# Autodesk Inventor assembly: Drivebase AM14U4 Square 28inx28in
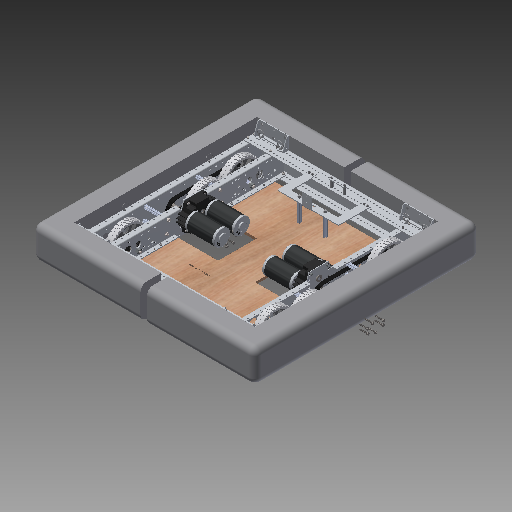
[picture p0: Inventor's stored thumbnail of the model, 512x512]
Saved by Autodesk Inventor 2018 (Build 220112000, 112)
## iProperties
Created: 2018-10-11
Part Number: Drivebase AM14U4 Square 28inx28in
Description: STEP AP214
Document SubType Name: Assembly
Designer: maste
Sending System: SolidWorks 2018
Preprocessor: SwSTEP 2.0
Title: AM14U4 Square.STEP
Revision Number: ANY
## Documents named in this file (10)
- \\studenthome\students\S-2513225\GitHub\2020CAD\Drivebase AM14U1\Main Assembly File\Drivebase AM14U4 Square 28inx28in.iam
- \\studenthome\students\S-2513225\GitHub\2020CAD\Drivebase AM14U1\Part Files\AM14U4 Square Half.iam
- \\studenthome\students\S-2513225\GitHub\2020CAD\Drivebase AM14U1\Part Files\Placeholder Belly Pan.ipt
- \\studenthome\students\S-2513225\GitHub\2020CAD\Drivebase AM14U1\Part Files\Bolts\92196A247_18-8 STAINLESS STEEL SOCKET HEAD CAP SCREW.ipt
- \\studenthome\students\S-2513225\GitHub\2020CAD\Drivebase AM14U1\Part Files\Locknuts\91831A011_TYPE 18-8 STAINLESS STL NYLON-INSERT LOCKNUT.ipt
- \\studenthome\students\S-2513225\GitHub\2020CAD\Drivebase AM14U1\Part Files\10-24 Washer.ipt
- \\studenthome\students\S-2513225\GitHub\2020CAD\Bumpers\Main Assembly File\Bumper Assembly.iam
- \\studenthome\students\S-2513225\GitHub\2020CAD\Bumpers\Part Files\95335A503_METRIC QUICK-RELEASE PIN.ipt
- \\studenthome\students\S-2513225\GitHub\2020CAD\Drivebase AM14U1\Part Files\Battery holder assembly.iam
- \\studenthome\students\S-2513225\GitHub\2020CAD\Drivebase AM14U1\Part Files\Strap mount.iam
## Components (43 placed, 10 different names)
1. AM14U4 Square Half_1 [sub-assembly] — Mate:1, Mate:2, Flush:1, Mate:3, Mate:4, Mate:5, Mate:8, Mate:9, Mate:12, Mate:13, Mate:14, Mate:15, Mate:20, Mate:21, Mate:54, Mate:55, Mate:56, Mate:57, Mate:58, Mate:66, Mate:67, Tangent:7, Tangent:8, Rotation:31, Rotation:32, Mate:72, Mate:73, Mate:74, Mate:75, Mate:76, Mate:77
2. AM14U4 Square Half_2 [sub-assembly] — Mate:1, Mate:2, Flush:1, Mate:6, Mate:7, Mate:10, Mate:11, Mate:16, Mate:17, Mate:18, Mate:19, Mate:59, Mate:60, Tangent:1, Mate:61, Tangent:2, Rotation:25, Rotation:26
3. Placeholder Belly Pan:1 — Mate:3, Mate:4, Mate:5, Mate:22, Mate:23, Mate:24, Mate:25, Mate:26, Mate:27, Mate:28, Mate:29, Rotation:1, Rotation:2, Rotation:3, Rotation:4, Rotation:5, Rotation:6, Rotation:7, Rotation:8, Rotation:9, Rotation:10, Rotation:11, Rotation:12, Rotation:13, Rotation:14, Rotation:15, Rotation:16, Mate:38, Mate:39, Mate:40, Mate:41, Mate:42, Mate:43, Mate:44, Mate:45
4. 92196A247_18-8 STAINLESS STEEL SOCKET HEAD CAP SCREW:1 — Mate:7, Mate:19, Mate:35, Rotation:5, Mate:50, Rotation:17
5. 92196A247_18-8 STAINLESS STEEL SOCKET HEAD CAP SCREW:2 — Mate:6, Mate:18, Mate:34, Rotation:7, Mate:51, Rotation:18
6. 92196A247_18-8 STAINLESS STEEL SOCKET HEAD CAP SCREW:3 — Mate:10, Mate:17, Mate:33, Rotation:9, Mate:52, Rotation:24
7. 92196A247_18-8 STAINLESS STEEL SOCKET HEAD CAP SCREW:4 — Mate:11, Mate:16, Mate:32, Rotation:11, Mate:53, Rotation:23
8. 92196A247_18-8 STAINLESS STEEL SOCKET HEAD CAP SCREW:5 — Mate:12, Mate:14, Mate:31, Rotation:13, Mate:46, Rotation:22
9. 92196A247_18-8 STAINLESS STEEL SOCKET HEAD CAP SCREW:6 — Mate:13, Mate:15, Mate:30, Rotation:15, Mate:47, Rotation:21
10. 92196A247_18-8 STAINLESS STEEL SOCKET HEAD CAP SCREW:7 — Mate:8, Mate:20, Mate:37, Rotation:1, Mate:48, Rotation:19
11. 92196A247_18-8 STAINLESS STEEL SOCKET HEAD CAP SCREW:8 — Mate:9, Mate:21, Mate:36, Rotation:3, Mate:49, Rotation:20
12. 91831A011_TYPE 18-8 STAINLESS STL NYLON-INSERT LOCKNUT:1 — Mate:42, Mate:49, Rotation:20
13. 91831A011_TYPE 18-8 STAINLESS STL NYLON-INSERT LOCKNUT:2 — Mate:43, Mate:48, Rotation:19
14. 91831A011_TYPE 18-8 STAINLESS STL NYLON-INSERT LOCKNUT:3 — Mate:44, Mate:47, Rotation:21
15. 91831A011_TYPE 18-8 STAINLESS STL NYLON-INSERT LOCKNUT:4 — Mate:45, Mate:46, Rotation:22
16. 91831A011_TYPE 18-8 STAINLESS STL NYLON-INSERT LOCKNUT:5 — Mate:41, Mate:53, Rotation:23
17. 91831A011_TYPE 18-8 STAINLESS STL NYLON-INSERT LOCKNUT:6 — Mate:40, Mate:52, Rotation:24
18. 91831A011_TYPE 18-8 STAINLESS STL NYLON-INSERT LOCKNUT:7 — Mate:39, Mate:51, Rotation:18
19. 91831A011_TYPE 18-8 STAINLESS STL NYLON-INSERT LOCKNUT:8 — Mate:38, Mate:50, Rotation:17
20. 10-24 Washer:1 — Mate:24, Mate:35, Rotation:6
21. 10-24 Washer:2 — Mate:25, Mate:34, Rotation:8
22. 10-24 Washer:3 — Mate:26, Mate:33, Rotation:10
23. 10-24 Washer:4 — Mate:27, Mate:32, Rotation:12
24. 10-24 Washer:5 — Mate:28, Mate:31, Rotation:14
25. 10-24 Washer:6 — Mate:29, Mate:30, Rotation:16
26. 10-24 Washer:7 — Mate:23, Mate:37, Rotation:2
27. 10-24 Washer:8 — Mate:22, Mate:36, Rotation:4
28. Bumper Assembly:1 [sub-assembly] — Mate:54, Mate:55, Mate:56, Mate:64, Mate:65, Mate:70, Mate:71, Tangent:5, Tangent:6, Tangent:9, Tangent:10, Rotation:29, Rotation:30, Rotation:33, Rotation:34
29. Bumper Assembly:2 [sub-assembly] — Mate:57, Mate:58, Mate:59, Mate:62, Mate:63, Mate:68, Mate:69, Tangent:3, Tangent:4, Tangent:11, Tangent:12, Rotation:27, Rotation:28, Rotation:35, Rotation:36
30. 95335A503_METRIC QUICK-RELEASE PIN:1 — Mate:62, Tangent:3, Rotation:27
31. 95335A503_METRIC QUICK-RELEASE PIN:2 — Mate:63, Tangent:4, Rotation:28
32. 95335A503_METRIC QUICK-RELEASE PIN:3 — Mate:65, Tangent:6, Rotation:30
33. 95335A503_METRIC QUICK-RELEASE PIN:4 — Mate:64, Tangent:5, Rotation:29
34. 95335A503_METRIC QUICK-RELEASE PIN:5 — Mate:71, Tangent:9, Rotation:33
35. 95335A503_METRIC QUICK-RELEASE PIN:6 — Mate:70, Tangent:10, Rotation:34
36. 95335A503_METRIC QUICK-RELEASE PIN:7 — Mate:69, Tangent:11, Rotation:35
37. 95335A503_METRIC QUICK-RELEASE PIN:8 — Mate:68, Tangent:12, Rotation:36
38. 95335A503_METRIC QUICK-RELEASE PIN:9 — Mate:61, Tangent:2, Rotation:26
39. 95335A503_METRIC QUICK-RELEASE PIN:10 — Mate:60, Tangent:1, Rotation:25
40. 95335A503_METRIC QUICK-RELEASE PIN:11 — Mate:66, Tangent:7, Rotation:31
41. 95335A503_METRIC QUICK-RELEASE PIN:12 — Mate:67, Tangent:8, Rotation:32
42. Battery holder assembly:1 [sub-assembly] — Mate:72, Mate:73, Mate:74
43. Strap mount:1 [sub-assembly] — Mate:75, Mate:76, Mate:77
## Relationships (126: Mate 77, RelateRotation 36, Tangent 12, Flush 1)
- Mate:1: AM14U4 Square Half_1 ↔ AM14U4 Square Half_2
- Mate:2: AM14U4 Square Half_1 ↔ AM14U4 Square Half_2
- Flush:1: AM14U4 Square Half_1 ↔ AM14U4 Square Half_2
- Mate:3: AM14U4 Square Half_1 ↔ Placeholder Belly Pan:1
- Mate:4: AM14U4 Square Half_1 ↔ Placeholder Belly Pan:1
- Mate:5: AM14U4 Square Half_1 ↔ Placeholder Belly Pan:1
- Mate:6: AM14U4 Square Half_2 ↔ 92196A247_18-8 STAINLESS STEEL SOCKET HEAD CAP SCREW:2
- Mate:7: AM14U4 Square Half_2 ↔ 92196A247_18-8 STAINLESS STEEL SOCKET HEAD CAP SCREW:1
- Mate:8: AM14U4 Square Half_1 ↔ 92196A247_18-8 STAINLESS STEEL SOCKET HEAD CAP SCREW:7
- Mate:9: AM14U4 Square Half_1 ↔ 92196A247_18-8 STAINLESS STEEL SOCKET HEAD CAP SCREW:8
- Mate:10: AM14U4 Square Half_2 ↔ 92196A247_18-8 STAINLESS STEEL SOCKET HEAD CAP SCREW:3
- Mate:11: AM14U4 Square Half_2 ↔ 92196A247_18-8 STAINLESS STEEL SOCKET HEAD CAP SCREW:4
- Mate:12: AM14U4 Square Half_1 ↔ 92196A247_18-8 STAINLESS STEEL SOCKET HEAD CAP SCREW:5
- Mate:13: AM14U4 Square Half_1 ↔ 92196A247_18-8 STAINLESS STEEL SOCKET HEAD CAP SCREW:6
- Mate:14: AM14U4 Square Half_1 ↔ 92196A247_18-8 STAINLESS STEEL SOCKET HEAD CAP SCREW:5
- Mate:15: AM14U4 Square Half_1 ↔ 92196A247_18-8 STAINLESS STEEL SOCKET HEAD CAP SCREW:6
- Mate:16: AM14U4 Square Half_2 ↔ 92196A247_18-8 STAINLESS STEEL SOCKET HEAD CAP SCREW:4
- Mate:17: AM14U4 Square Half_2 ↔ 92196A247_18-8 STAINLESS STEEL SOCKET HEAD CAP SCREW:3
- Mate:18: AM14U4 Square Half_2 ↔ 92196A247_18-8 STAINLESS STEEL SOCKET HEAD CAP SCREW:2
- Mate:19: AM14U4 Square Half_2 ↔ 92196A247_18-8 STAINLESS STEEL SOCKET HEAD CAP SCREW:1
- Mate:20: AM14U4 Square Half_1 ↔ 92196A247_18-8 STAINLESS STEEL SOCKET HEAD CAP SCREW:7
- Mate:21: AM14U4 Square Half_1 ↔ 92196A247_18-8 STAINLESS STEEL SOCKET HEAD CAP SCREW:8
- Mate:22: Placeholder Belly Pan:1 ↔ 10-24 Washer:8
- Mate:23: Placeholder Belly Pan:1 ↔ 10-24 Washer:7
- Mate:24: Placeholder Belly Pan:1 ↔ 10-24 Washer:1
- Mate:25: Placeholder Belly Pan:1 ↔ 10-24 Washer:2
- Mate:26: Placeholder Belly Pan:1 ↔ 10-24 Washer:3
- Mate:27: Placeholder Belly Pan:1 ↔ 10-24 Washer:4
- Mate:28: Placeholder Belly Pan:1 ↔ 10-24 Washer:5
- Mate:29: Placeholder Belly Pan:1 ↔ 10-24 Washer:6
- Mate:30: 92196A247_18-8 STAINLESS STEEL SOCKET HEAD CAP SCREW:6 ↔ 10-24 Washer:6
- Mate:31: 92196A247_18-8 STAINLESS STEEL SOCKET HEAD CAP SCREW:5 ↔ 10-24 Washer:5
- Mate:32: 92196A247_18-8 STAINLESS STEEL SOCKET HEAD CAP SCREW:4 ↔ 10-24 Washer:4
- Mate:33: 92196A247_18-8 STAINLESS STEEL SOCKET HEAD CAP SCREW:3 ↔ 10-24 Washer:3
- Mate:34: 92196A247_18-8 STAINLESS STEEL SOCKET HEAD CAP SCREW:2 ↔ 10-24 Washer:2
- Mate:35: 92196A247_18-8 STAINLESS STEEL SOCKET HEAD CAP SCREW:1 ↔ 10-24 Washer:1
- Mate:36: 92196A247_18-8 STAINLESS STEEL SOCKET HEAD CAP SCREW:8 ↔ 10-24 Washer:8
- Mate:37: 92196A247_18-8 STAINLESS STEEL SOCKET HEAD CAP SCREW:7 ↔ 10-24 Washer:7
- Rotation:1 [RelateRotation] (1 ul): Placeholder Belly Pan:1 ↔ 92196A247_18-8 STAINLESS STEEL SOCKET HEAD CAP SCREW:7
- Rotation:2 [RelateRotation] (1 ul): Placeholder Belly Pan:1 ↔ 10-24 Washer:7
- Rotation:3 [RelateRotation] (1 ul): Placeholder Belly Pan:1 ↔ 92196A247_18-8 STAINLESS STEEL SOCKET HEAD CAP SCREW:8
- Rotation:4 [RelateRotation] (1 ul): Placeholder Belly Pan:1 ↔ 10-24 Washer:8
- Rotation:5 [RelateRotation] (1 ul): Placeholder Belly Pan:1 ↔ 92196A247_18-8 STAINLESS STEEL SOCKET HEAD CAP SCREW:1
- Rotation:6 [RelateRotation] (1 ul): Placeholder Belly Pan:1 ↔ 10-24 Washer:1
- Rotation:7 [RelateRotation] (1 ul): Placeholder Belly Pan:1 ↔ 92196A247_18-8 STAINLESS STEEL SOCKET HEAD CAP SCREW:2
- Rotation:8 [RelateRotation] (1 ul): Placeholder Belly Pan:1 ↔ 10-24 Washer:2
- Rotation:9 [RelateRotation] (1 ul): Placeholder Belly Pan:1 ↔ 92196A247_18-8 STAINLESS STEEL SOCKET HEAD CAP SCREW:3
- Rotation:10 [RelateRotation] (1 ul): Placeholder Belly Pan:1 ↔ 10-24 Washer:3
- Rotation:11 [RelateRotation] (1 ul): Placeholder Belly Pan:1 ↔ 92196A247_18-8 STAINLESS STEEL SOCKET HEAD CAP SCREW:4
- Rotation:12 [RelateRotation] (1 ul): Placeholder Belly Pan:1 ↔ 10-24 Washer:4
- Rotation:13 [RelateRotation] (1 ul): Placeholder Belly Pan:1 ↔ 92196A247_18-8 STAINLESS STEEL SOCKET HEAD CAP SCREW:5
- Rotation:14 [RelateRotation] (1 ul): Placeholder Belly Pan:1 ↔ 10-24 Washer:5
- Rotation:15 [RelateRotation] (1 ul): Placeholder Belly Pan:1 ↔ 92196A247_18-8 STAINLESS STEEL SOCKET HEAD CAP SCREW:6
- Rotation:16 [RelateRotation] (1 ul): Placeholder Belly Pan:1 ↔ 10-24 Washer:6
- Mate:38: Placeholder Belly Pan:1 ↔ 91831A011_TYPE 18-8 STAINLESS STL NYLON-INSERT LOCKNUT:8
- Mate:39: Placeholder Belly Pan:1 ↔ 91831A011_TYPE 18-8 STAINLESS STL NYLON-INSERT LOCKNUT:7
- Mate:40: Placeholder Belly Pan:1 ↔ 91831A011_TYPE 18-8 STAINLESS STL NYLON-INSERT LOCKNUT:6
- Mate:41: Placeholder Belly Pan:1 ↔ 91831A011_TYPE 18-8 STAINLESS STL NYLON-INSERT LOCKNUT:5
- Mate:42: Placeholder Belly Pan:1 ↔ 91831A011_TYPE 18-8 STAINLESS STL NYLON-INSERT LOCKNUT:1
- Mate:43: Placeholder Belly Pan:1 ↔ 91831A011_TYPE 18-8 STAINLESS STL NYLON-INSERT LOCKNUT:2
- Mate:44: Placeholder Belly Pan:1 ↔ 91831A011_TYPE 18-8 STAINLESS STL NYLON-INSERT LOCKNUT:3
- Mate:45: Placeholder Belly Pan:1 ↔ 91831A011_TYPE 18-8 STAINLESS STL NYLON-INSERT LOCKNUT:4
- Mate:46: 92196A247_18-8 STAINLESS STEEL SOCKET HEAD CAP SCREW:5 ↔ 91831A011_TYPE 18-8 STAINLESS STL NYLON-INSERT LOCKNUT:4
- Mate:47: 92196A247_18-8 STAINLESS STEEL SOCKET HEAD CAP SCREW:6 ↔ 91831A011_TYPE 18-8 STAINLESS STL NYLON-INSERT LOCKNUT:3
- Mate:48: 92196A247_18-8 STAINLESS STEEL SOCKET HEAD CAP SCREW:7 ↔ 91831A011_TYPE 18-8 STAINLESS STL NYLON-INSERT LOCKNUT:2
- Mate:49: 92196A247_18-8 STAINLESS STEEL SOCKET HEAD CAP SCREW:8 ↔ 91831A011_TYPE 18-8 STAINLESS STL NYLON-INSERT LOCKNUT:1
- Mate:50: 92196A247_18-8 STAINLESS STEEL SOCKET HEAD CAP SCREW:1 ↔ 91831A011_TYPE 18-8 STAINLESS STL NYLON-INSERT LOCKNUT:8
- Mate:51: 92196A247_18-8 STAINLESS STEEL SOCKET HEAD CAP SCREW:2 ↔ 91831A011_TYPE 18-8 STAINLESS STL NYLON-INSERT LOCKNUT:7
- Mate:52: 92196A247_18-8 STAINLESS STEEL SOCKET HEAD CAP SCREW:3 ↔ 91831A011_TYPE 18-8 STAINLESS STL NYLON-INSERT LOCKNUT:6
- Mate:53: 92196A247_18-8 STAINLESS STEEL SOCKET HEAD CAP SCREW:4 ↔ 91831A011_TYPE 18-8 STAINLESS STL NYLON-INSERT LOCKNUT:5
- Rotation:17 [RelateRotation] (1 ul): 92196A247_18-8 STAINLESS STEEL SOCKET HEAD CAP SCREW:1 ↔ 91831A011_TYPE 18-8 STAINLESS STL NYLON-INSERT LOCKNUT:8
- Rotation:18 [RelateRotation] (1 ul): 92196A247_18-8 STAINLESS STEEL SOCKET HEAD CAP SCREW:2 ↔ 91831A011_TYPE 18-8 STAINLESS STL NYLON-INSERT LOCKNUT:7
- Rotation:19 [RelateRotation] (1 ul): 92196A247_18-8 STAINLESS STEEL SOCKET HEAD CAP SCREW:7 ↔ 91831A011_TYPE 18-8 STAINLESS STL NYLON-INSERT LOCKNUT:2
- Rotation:20 [RelateRotation] (1 ul): 92196A247_18-8 STAINLESS STEEL SOCKET HEAD CAP SCREW:8 ↔ 91831A011_TYPE 18-8 STAINLESS STL NYLON-INSERT LOCKNUT:1
- Rotation:21 [RelateRotation] (1 ul): 92196A247_18-8 STAINLESS STEEL SOCKET HEAD CAP SCREW:6 ↔ 91831A011_TYPE 18-8 STAINLESS STL NYLON-INSERT LOCKNUT:3
- Rotation:22 [RelateRotation] (1 ul): 92196A247_18-8 STAINLESS STEEL SOCKET HEAD CAP SCREW:5 ↔ 91831A011_TYPE 18-8 STAINLESS STL NYLON-INSERT LOCKNUT:4
- Rotation:23 [RelateRotation] (1 ul): 92196A247_18-8 STAINLESS STEEL SOCKET HEAD CAP SCREW:4 ↔ 91831A011_TYPE 18-8 STAINLESS STL NYLON-INSERT LOCKNUT:5
- Rotation:24 [RelateRotation] (1 ul): 92196A247_18-8 STAINLESS STEEL SOCKET HEAD CAP SCREW:3 ↔ 91831A011_TYPE 18-8 STAINLESS STL NYLON-INSERT LOCKNUT:6
- Mate:54: AM14U4 Square Half_1 ↔ Bumper Assembly:1
- Mate:55: AM14U4 Square Half_1 ↔ Bumper Assembly:1
- Mate:56: AM14U4 Square Half_1 ↔ Bumper Assembly:1
- Mate:57: AM14U4 Square Half_1 ↔ Bumper Assembly:2
- Mate:58: AM14U4 Square Half_1 ↔ Bumper Assembly:2
- Mate:59: AM14U4 Square Half_2 ↔ Bumper Assembly:2
- Mate:60: AM14U4 Square Half_2 ↔ 95335A503_METRIC QUICK-RELEASE PIN:10
- Tangent:1: AM14U4 Square Half_2 ↔ 95335A503_METRIC QUICK-RELEASE PIN:10
- Mate:61: AM14U4 Square Half_2 ↔ 95335A503_METRIC QUICK-RELEASE PIN:9
- Mate:62: Bumper Assembly:2 ↔ 95335A503_METRIC QUICK-RELEASE PIN:1
- Mate:63: Bumper Assembly:2 ↔ 95335A503_METRIC QUICK-RELEASE PIN:2
- Mate:64: Bumper Assembly:1 ↔ 95335A503_METRIC QUICK-RELEASE PIN:4
- Mate:65: Bumper Assembly:1 ↔ 95335A503_METRIC QUICK-RELEASE PIN:3
- Mate:66: AM14U4 Square Half_1 ↔ 95335A503_METRIC QUICK-RELEASE PIN:11
- Mate:67: AM14U4 Square Half_1 ↔ 95335A503_METRIC QUICK-RELEASE PIN:12
- Mate:68: Bumper Assembly:2 ↔ 95335A503_METRIC QUICK-RELEASE PIN:8
- Mate:69: Bumper Assembly:2 ↔ 95335A503_METRIC QUICK-RELEASE PIN:7
- Mate:70: Bumper Assembly:1 ↔ 95335A503_METRIC QUICK-RELEASE PIN:6
- Mate:71: Bumper Assembly:1 ↔ 95335A503_METRIC QUICK-RELEASE PIN:5
- Tangent:2: AM14U4 Square Half_2 ↔ 95335A503_METRIC QUICK-RELEASE PIN:9
- Tangent:3: Bumper Assembly:2 ↔ 95335A503_METRIC QUICK-RELEASE PIN:1
- Tangent:4: Bumper Assembly:2 ↔ 95335A503_METRIC QUICK-RELEASE PIN:2
- Tangent:5: Bumper Assembly:1 ↔ 95335A503_METRIC QUICK-RELEASE PIN:4
- Tangent:6: Bumper Assembly:1 ↔ 95335A503_METRIC QUICK-RELEASE PIN:3
- Tangent:7: AM14U4 Square Half_1 ↔ 95335A503_METRIC QUICK-RELEASE PIN:11
- Tangent:8: AM14U4 Square Half_1 ↔ 95335A503_METRIC QUICK-RELEASE PIN:12
- Tangent:9: Bumper Assembly:1 ↔ 95335A503_METRIC QUICK-RELEASE PIN:5
- Tangent:10: Bumper Assembly:1 ↔ 95335A503_METRIC QUICK-RELEASE PIN:6
- Tangent:11: Bumper Assembly:2 ↔ 95335A503_METRIC QUICK-RELEASE PIN:7
- Tangent:12: Bumper Assembly:2 ↔ 95335A503_METRIC QUICK-RELEASE PIN:8
- Rotation:25 [RelateRotation] (1 ul): AM14U4 Square Half_2 ↔ 95335A503_METRIC QUICK-RELEASE PIN:10
- Rotation:26 [RelateRotation] (1 ul): AM14U4 Square Half_2 ↔ 95335A503_METRIC QUICK-RELEASE PIN:9
- Rotation:27 [RelateRotation] (1 ul): Bumper Assembly:2 ↔ 95335A503_METRIC QUICK-RELEASE PIN:1
- Rotation:28 [RelateRotation] (1 ul): Bumper Assembly:2 ↔ 95335A503_METRIC QUICK-RELEASE PIN:2
- Rotation:29 [RelateRotation] (1 ul): Bumper Assembly:1 ↔ 95335A503_METRIC QUICK-RELEASE PIN:4
- Rotation:30 [RelateRotation] (1 ul): Bumper Assembly:1 ↔ 95335A503_METRIC QUICK-RELEASE PIN:3
- Rotation:31 [RelateRotation] (1 ul): AM14U4 Square Half_1 ↔ 95335A503_METRIC QUICK-RELEASE PIN:11
- Rotation:32 [RelateRotation] (1 ul): AM14U4 Square Half_1 ↔ 95335A503_METRIC QUICK-RELEASE PIN:12
- Rotation:33 [RelateRotation] (1 ul): Bumper Assembly:1 ↔ 95335A503_METRIC QUICK-RELEASE PIN:5
- Rotation:34 [RelateRotation] (1 ul): Bumper Assembly:1 ↔ 95335A503_METRIC QUICK-RELEASE PIN:6
- Rotation:35 [RelateRotation] (1 ul): Bumper Assembly:2 ↔ 95335A503_METRIC QUICK-RELEASE PIN:7
- Rotation:36 [RelateRotation] (1 ul): Bumper Assembly:2 ↔ 95335A503_METRIC QUICK-RELEASE PIN:8
- Mate:72: AM14U4 Square Half_1 ↔ Battery holder assembly:1
- Mate:73: AM14U4 Square Half_1 ↔ Battery holder assembly:1
- Mate:74: AM14U4 Square Half_1 ↔ Battery holder assembly:1
- Mate:75: AM14U4 Square Half_1 ↔ Strap mount:1
- Mate:76: AM14U4 Square Half_1 ↔ Strap mount:1
- Mate:77: AM14U4 Square Half_1 ↔ Strap mount:1
